# Autodesk Inventor assembly: MontagemPneuRoda
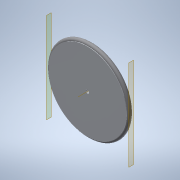
[picture p0: Inventor's stored thumbnail of the model, 180x180]
Saved by Autodesk Inventor 2021 (Build 250183000, 183)
## iProperties
Created: 2020-05-19
Part Number: MontagemPneuRoda
Material: Genérico
Document SubType Name: Assembly
Designer: Mathe
Mass: 43.4 g
Surface Area: 106.898 cm^2
Volume: 16.7658 cm^3
Density: 2.5886 g/cm^3
Author: Mathe
## Documents named in this file (3)
- D:\Projetos\Robo_TCC\MontagemPneuRoda.iam
- D:\Projetos\Robo_TCC\pneu_com_piso.ipt
- D:\Projetos\Robo_TCC\roda aluminio oring.ipt
## Components (2 placed, 2 different names)
1. roda aluminio oring:1 — Coincidência:1
2. pneu_com_piso:1 — Coincidência:1
## Relationships (1: Mate 1)
- Coincidência:1 [Mate]: roda aluminio oring:1 ↔ pneu_com_piso:1
